# Autodesk Inventor assembly: Stepper_Motor_Assembly
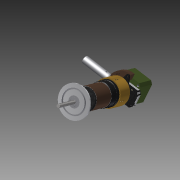
[picture p0: Inventor's stored thumbnail of the model, 180x180]
Saved by Autodesk Inventor 2014 (Build 180170000, 170)
## iProperties
Created: 2014-11-07
Part Number: Stepper_Motor_Assembly
Document SubType Name: Assembly
Designer: nfitch
Author: nfitch
## Documents named in this file (7)
- C:\Users\nfitch\Desktop\Stepper_Motor_Parts\Stepper_Motor_Assembly.iam
- C:\Users\nfitch\Desktop\Stepper_Motor_Parts\AMT102_Wide.ipt
- C:\Users\nfitch\Desktop\Stepper_Motor_Parts\Stepper_Motor.ipt
- C:\Users\nfitch\Desktop\Stepper_Motor_Parts\Mount.ipt
- C:\Users\nfitch\Desktop\Stepper_Motor_Parts\Coupler.ipt
- C:\Users\nfitch\Desktop\Stepper_Motor_Parts\670022.ipt
- C:\Users\nfitch\Desktop\Stepper_Motor_Parts\TR50_M-Step.ipt
## Components (6 placed, 6 different names)
1. AMT102_Wide:1 — Mate:4, Mate:5, Mate:6, Mate:8
2. Stepper_Motor:1 — Mate:2, Mate:3, Mate:4, Angle:1, Mate:7, Angle:2
3. Mount:1 — Mate:2, Mate:3, Mate:5, Angle:1, Mate:6, Mate:11, Mate:12
4. Coupler:1 — Mate:7, Angle:2, Mate:8, Mate:9, Mate:10
5. 670022:1 — Mate:9, Mate:10
6. TR50_M-Step:1 — Mate:11, Mate:12
## Relationships (13: Mate 11, Angle 2)
- Mate:2: Stepper_Motor:1 ↔ Mount:1
- Mate:3: Stepper_Motor:1 ↔ Mount:1
- Mate:4: AMT102_Wide:1 ↔ Stepper_Motor:1
- Mate:5: AMT102_Wide:1 ↔ Mount:1
- Angle:1 (0 deg): Stepper_Motor:1 ↔ Mount:1
- Mate:6 (-0.25 mm): AMT102_Wide:1 ↔ Mount:1
- Mate:7: Stepper_Motor:1 ↔ Coupler:1
- Angle:2 (0 deg): Stepper_Motor:1 ↔ Coupler:1
- Mate:8: AMT102_Wide:1 ↔ Coupler:1
- Mate:9: Coupler:1 ↔ 670022:1
- Mate:10 (2.5 mm): Coupler:1 ↔ 670022:1
- Mate:11: Mount:1 ↔ TR50_M-Step:1
- Mate:12: Mount:1 ↔ TR50_M-Step:1
